# Autodesk Inventor assembly: Wear P
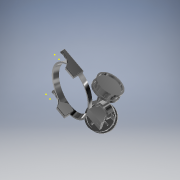
[picture p0: Inventor's stored thumbnail of the model, 180x180]
Saved by Autodesk Inventor 2021 (Build 250183000, 183)
## iProperties
Created: 2021-05-30
Part Number: Wear P
Document SubType Name: Assembly
Designer: AHUJA
Author: AHUJA
## Documents named in this file (3)
- F:\Files\ODM GEAR IPT\My worl\Wear P.iam
- F:\Files\ODM GEAR IPT\My worl\Gas Propulsion.ipt
- F:\Files\ODM GEAR IPT\My worl\Wire Attachement.ipt
## Components (3 placed, 2 different names)
1. Gas Propulsion:1 — Flush:1, Flush:2, Mate:2, Angle:1, Flush:3
2. Wire Attachement:1 — Flush:3, Mate:3, Flush:4, Flush:5
3. Wire Attachement:2 — Flush:1, Mate:1, Flush:4, Flush:5
## Relationships (9: Flush 5, Mate 3, Angle 1)
- Flush:1: Gas Propulsion:1 ↔ Wire Attachement:2
- Flush:2 (46 mm): Gas Propulsion:1
- Mate:1: Wire Attachement:2
- Mate:2: Gas Propulsion:1
- Angle:1 (0 deg): Gas Propulsion:1
- Flush:3: Gas Propulsion:1 ↔ Wire Attachement:1
- Mate:3 (2 mm): Wire Attachement:1
- Flush:4: Wire Attachement:1 ↔ Wire Attachement:2
- Flush:5: Wire Attachement:1 ↔ Wire Attachement:2
